# Autodesk Inventor assembly: model
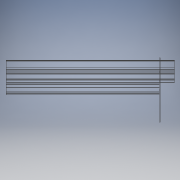
[picture p0: Inventor's stored thumbnail of the model, 180x180]
Saved by Autodesk Inventor 2018.2 (Build 222227000, 227)
## iProperties
Created: 2018-02-25
Part Number: model
Material: 一般
Document SubType Name: Assembly
Designer: ku_sk
Author: ku_sk
## Documents named in this file (4)
- C:\Users\ku_sk\Documents\Inventor\AeroCAD2018\設計\Rr.wing\model.iam
- C:\Users\ku_sk\Documents\Inventor\AeroCAD2018\設計\Rr.wing\parts\main frap.ipt
- C:\Users\ku_sk\Documents\Inventor\AeroCAD2018\設計\Rr.wing\parts\endplate.ipt
- C:\Users\ku_sk\Documents\Inventor\AeroCAD2018\設計\Rr.wing\parts\subflap.ipt
## Components (5 placed, 3 different names)
1. endplate:1 — メイト:1, フラッシュ:2, メイト:5, メイト:6, メイト:7, メイト:8
2. endplate:2 — メイト:2, 角度:1, フラッシュ:2, メイト:4, メイト:9
3. main frap:1 — フラッシュ:1, メイト:1, メイト:2, 角度:2, メイト:3, メイト:4, メイト:5, 角度:3
4. subflap:1 — メイト:6, メイト:7, 角度:3, 角度:4
5. subflap:2 — メイト:8, メイト:9, 角度:4
## Relationships (15: Mate 9, Angle 4, Flush 2)
- フラッシュ:1 [Flush]: main frap:1
- メイト:1 [Mate]: endplate:1 ↔ main frap:1
- メイト:2 [Mate]: endplate:2 ↔ main frap:1
- 角度:1 [Angle] (0 deg): endplate:2
- フラッシュ:2 [Flush]: endplate:1 ↔ endplate:2
- 角度:2 [Angle] (-15 deg): main frap:1
- メイト:3 [Mate]: main frap:1
- メイト:4 [Mate]: endplate:2 ↔ main frap:1
- メイト:5 [Mate]: endplate:1 ↔ main frap:1
- メイト:6 [Mate]: endplate:1 ↔ subflap:1
- メイト:7 [Mate]: endplate:1 ↔ subflap:1
- 角度:3 [Angle] (-15 deg): main frap:1 ↔ subflap:1
- メイト:8 [Mate]: endplate:1 ↔ subflap:2
- メイト:9 [Mate]: endplate:2 ↔ subflap:2
- 角度:4 [Angle] (-15 deg): subflap:1 ↔ subflap:2
